(part 1 of 2)
# Autodesk Inventor assembly: carrier_board_2019-06-12
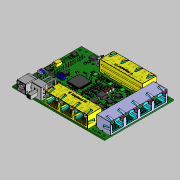
[picture p0: Inventor's stored thumbnail of the model, 180x180]
Saved by Autodesk Inventor 2020 (Build 240168000, 168)
## iProperties
Company: Open CASCADE
Created: 2019-06-12
Part Number: carrier_board_2019-06-12
Description: Open CASCADE Model
Document SubType Name: Assembly
Designer: Varga Daniel
Authority: Unknown
Title: Open CASCADE Shape Model
Author: Author
Sending System: Open CASCADE 6.8
Preprocessor: Open CASCADE STEP processor 6.8
## Documents named in this file (428)
- C:\!_Dani\!_cloud\OneDrive\!_munka\Revolution\StructuralParts\Brain\Inventor imported\BRpcbA\carrier_board_2019-06-12.iam
- C:\!_Dani\!_cloud\OneDrive\!_munka\Revolution\StructuralParts\Brain\Inventor imported\BRpcbA\Board.iam
- C:\!_Dani\!_cloud\OneDrive\!_munka\Revolution\StructuralParts\Brain\Inventor imported\BRpcbA\R177.iam
- C:\!_Dani\!_cloud\OneDrive\!_munka\Revolution\StructuralParts\Brain\Inventor imported\BRpcbA\CON1.iam
- C:\!_Dani\!_cloud\OneDrive\!_munka\Revolution\StructuralParts\Brain\Inventor imported\BRpcbA\R81.iam
- C:\!_Dani\!_cloud\OneDrive\!_munka\Revolution\StructuralParts\Brain\Inventor imported\BRpcbA\C45.iam
- C:\!_Dani\!_cloud\OneDrive\!_munka\Revolution\StructuralParts\Brain\Inventor imported\BRpcbA\U4.iam
- C:\!_Dani\!_cloud\OneDrive\!_munka\Revolution\StructuralParts\Brain\Inventor imported\BRpcbA\D37.iam
- C:\!_Dani\!_cloud\OneDrive\!_munka\Revolution\StructuralParts\Brain\Inventor imported\BRpcbA\D33.iam
- C:\!_Dani\!_cloud\OneDrive\!_munka\Revolution\StructuralParts\Brain\Inventor imported\BRpcbA\D32.iam
- C:\!_Dani\!_cloud\OneDrive\!_munka\Revolution\StructuralParts\Brain\Inventor imported\BRpcbA\C48.iam
- C:\!_Dani\!_cloud\OneDrive\!_munka\Revolution\StructuralParts\Brain\Inventor imported\BRpcbA\C47.iam
- C:\!_Dani\!_cloud\OneDrive\!_munka\Revolution\StructuralParts\Brain\Inventor imported\BRpcbA\D31.iam
- C:\!_Dani\!_cloud\OneDrive\!_munka\Revolution\StructuralParts\Brain\Inventor imported\BRpcbA\C46.iam
- C:\!_Dani\!_cloud\OneDrive\!_munka\Revolution\StructuralParts\Brain\Inventor imported\BRpcbA\R82.iam
- C:\!_Dani\!_cloud\OneDrive\!_munka\Revolution\StructuralParts\Brain\Inventor imported\BRpcbA\R26.iam
- C:\!_Dani\!_cloud\OneDrive\!_munka\Revolution\StructuralParts\Brain\Inventor imported\BRpcbA\C20.iam
- C:\!_Dani\!_cloud\OneDrive\!_munka\Revolution\StructuralParts\Brain\Inventor imported\BRpcbA\U2.iam
- C:\!_Dani\!_cloud\OneDrive\!_munka\Revolution\StructuralParts\Brain\Inventor imported\BRpcbA\D9.iam
- C:\!_Dani\!_cloud\OneDrive\!_munka\Revolution\StructuralParts\Brain\Inventor imported\BRpcbA\D5.iam
- C:\!_Dani\!_cloud\OneDrive\!_munka\Revolution\StructuralParts\Brain\Inventor imported\BRpcbA\D4.iam
- C:\!_Dani\!_cloud\OneDrive\!_munka\Revolution\StructuralParts\Brain\Inventor imported\BRpcbA\C23.iam
- C:\!_Dani\!_cloud\OneDrive\!_munka\Revolution\StructuralParts\Brain\Inventor imported\BRpcbA\C22.iam
- C:\!_Dani\!_cloud\OneDrive\!_munka\Revolution\StructuralParts\Brain\Inventor imported\BRpcbA\D1.iam
- C:\!_Dani\!_cloud\OneDrive\!_munka\Revolution\StructuralParts\Brain\Inventor imported\BRpcbA\C21.iam
- C:\!_Dani\!_cloud\OneDrive\!_munka\Revolution\StructuralParts\Brain\Inventor imported\BRpcbA\R27.iam
- C:\!_Dani\!_cloud\OneDrive\!_munka\Revolution\StructuralParts\Brain\Inventor imported\BRpcbA\R180.iam
- C:\!_Dani\!_cloud\OneDrive\!_munka\Revolution\StructuralParts\Brain\Inventor imported\BRpcbA\R109.iam
- C:\!_Dani\!_cloud\OneDrive\!_munka\Revolution\StructuralParts\Brain\Inventor imported\BRpcbA\R71.iam
- C:\!_Dani\!_cloud\OneDrive\!_munka\Revolution\StructuralParts\Brain\Inventor imported\BRpcbA\D72.iam
- C:\!_Dani\!_cloud\OneDrive\!_munka\Revolution\StructuralParts\Brain\Inventor imported\BRpcbA\Q4.iam
- C:\!_Dani\!_cloud\OneDrive\!_munka\Revolution\StructuralParts\Brain\Inventor imported\BRpcbA\R176.iam
- C:\!_Dani\!_cloud\OneDrive\!_munka\Revolution\StructuralParts\Brain\Inventor imported\BRpcbA\R175.iam
- C:\!_Dani\!_cloud\OneDrive\!_munka\Revolution\StructuralParts\Brain\Inventor imported\BRpcbA\R174.iam
- C:\!_Dani\!_cloud\OneDrive\!_munka\Revolution\StructuralParts\Brain\Inventor imported\BRpcbA\R173.iam
- C:\!_Dani\!_cloud\OneDrive\!_munka\Revolution\StructuralParts\Brain\Inventor imported\BRpcbA\R172.iam
- C:\!_Dani\!_cloud\OneDrive\!_munka\Revolution\StructuralParts\Brain\Inventor imported\BRpcbA\R171.iam
- C:\!_Dani\!_cloud\OneDrive\!_munka\Revolution\StructuralParts\Brain\Inventor imported\BRpcbA\R170.iam
- C:\!_Dani\!_cloud\OneDrive\!_munka\Revolution\StructuralParts\Brain\Inventor imported\BRpcbA\R169.iam
- C:\!_Dani\!_cloud\OneDrive\!_munka\Revolution\StructuralParts\Brain\Inventor imported\BRpcbA\R168.iam
- C:\!_Dani\!_cloud\OneDrive\!_munka\Revolution\StructuralParts\Brain\Inventor imported\BRpcbA\R167.iam
- C:\!_Dani\!_cloud\OneDrive\!_munka\Revolution\StructuralParts\Brain\Inventor imported\BRpcbA\R166.iam
- C:\!_Dani\!_cloud\OneDrive\!_munka\Revolution\StructuralParts\Brain\Inventor imported\BRpcbA\R165.iam
- C:\!_Dani\!_cloud\OneDrive\!_munka\Revolution\StructuralParts\Brain\Inventor imported\BRpcbA\R80.iam
- C:\!_Dani\!_cloud\OneDrive\!_munka\Revolution\StructuralParts\Brain\Inventor imported\BRpcbA\R79.iam
- C:\!_Dani\!_cloud\OneDrive\!_munka\Revolution\StructuralParts\Brain\Inventor imported\BRpcbA\R67.iam
- C:\!_Dani\!_cloud\OneDrive\!_munka\Revolution\StructuralParts\Brain\Inventor imported\BRpcbA\R66.iam
- C:\!_Dani\!_cloud\OneDrive\!_munka\Revolution\StructuralParts\Brain\Inventor imported\BRpcbA\R51.iam
- C:\!_Dani\!_cloud\OneDrive\!_munka\Revolution\StructuralParts\Brain\Inventor imported\BRpcbA\R50.iam
- C:\!_Dani\!_cloud\OneDrive\!_munka\Revolution\StructuralParts\Brain\Inventor imported\BRpcbA\R39.iam
- C:\!_Dani\!_cloud\OneDrive\!_munka\Revolution\StructuralParts\Brain\Inventor imported\BRpcbA\R38.iam
- C:\!_Dani\!_cloud\OneDrive\!_munka\Revolution\StructuralParts\Brain\Inventor imported\BRpcbA\R23.iam
- C:\!_Dani\!_cloud\OneDrive\!_munka\Revolution\StructuralParts\Brain\Inventor imported\BRpcbA\R22.iam
- C:\!_Dani\!_cloud\OneDrive\!_munka\Revolution\StructuralParts\Brain\Inventor imported\BRpcbA\R9.iam
- C:\!_Dani\!_cloud\OneDrive\!_munka\Revolution\StructuralParts\Brain\Inventor imported\BRpcbA\R8.iam
- C:\!_Dani\!_cloud\OneDrive\!_munka\Revolution\StructuralParts\Brain\Inventor imported\BRpcbA\FB1.iam
- C:\!_Dani\!_cloud\OneDrive\!_munka\Revolution\StructuralParts\Brain\Inventor imported\BRpcbA\C2.iam
- C:\!_Dani\!_cloud\OneDrive\!_munka\Revolution\StructuralParts\Brain\Inventor imported\BRpcbA\FU1.iam
- C:\!_Dani\!_cloud\OneDrive\!_munka\Revolution\StructuralParts\Brain\Inventor imported\BRpcbA\C97.iam
- C:\!_Dani\!_cloud\OneDrive\!_munka\Revolution\StructuralParts\Brain\Inventor imported\BRpcbA\U16.iam
- C:\!_Dani\!_cloud\OneDrive\!_munka\Revolution\StructuralParts\Brain\Inventor imported\BRpcbA\U14.iam
- C:\!_Dani\!_cloud\OneDrive\!_munka\Revolution\StructuralParts\Brain\Inventor imported\BRpcbA\U8.iam
- C:\!_Dani\!_cloud\OneDrive\!_munka\Revolution\StructuralParts\Brain\Inventor imported\BRpcbA\U6.iam
- C:\!_Dani\!_cloud\OneDrive\!_munka\Revolution\StructuralParts\Brain\Inventor imported\BRpcbA\R161.iam
- C:\!_Dani\!_cloud\OneDrive\!_munka\Revolution\StructuralParts\Brain\Inventor imported\BRpcbA\R150.iam
- C:\!_Dani\!_cloud\OneDrive\!_munka\Revolution\StructuralParts\Brain\Inventor imported\BRpcbA\R127.iam
- C:\!_Dani\!_cloud\OneDrive\!_munka\Revolution\StructuralParts\Brain\Inventor imported\BRpcbA\R118.iam
- C:\!_Dani\!_cloud\OneDrive\!_munka\Revolution\StructuralParts\Brain\Inventor imported\BRpcbA\R116.iam
- C:\!_Dani\!_cloud\OneDrive\!_munka\Revolution\StructuralParts\Brain\Inventor imported\BRpcbA\R115.iam
- C:\!_Dani\!_cloud\OneDrive\!_munka\Revolution\StructuralParts\Brain\Inventor imported\BRpcbA\R114.iam
- C:\!_Dani\!_cloud\OneDrive\!_munka\Revolution\StructuralParts\Brain\Inventor imported\BRpcbA\R111.iam
- C:\!_Dani\!_cloud\OneDrive\!_munka\Revolution\StructuralParts\Brain\Inventor imported\BRpcbA\R110.iam
- C:\!_Dani\!_cloud\OneDrive\!_munka\Revolution\StructuralParts\Brain\Inventor imported\BRpcbA\R106.iam
- C:\!_Dani\!_cloud\OneDrive\!_munka\Revolution\StructuralParts\Brain\Inventor imported\BRpcbA\R105.iam
- C:\!_Dani\!_cloud\OneDrive\!_munka\Revolution\StructuralParts\Brain\Inventor imported\BRpcbA\R99.iam
- C:\!_Dani\!_cloud\OneDrive\!_munka\Revolution\StructuralParts\Brain\Inventor imported\BRpcbA\R98.iam
- C:\!_Dani\!_cloud\OneDrive\!_munka\Revolution\StructuralParts\Brain\Inventor imported\BRpcbA\R95.iam
- C:\!_Dani\!_cloud\OneDrive\!_munka\Revolution\StructuralParts\Brain\Inventor imported\BRpcbA\R92.iam
- C:\!_Dani\!_cloud\OneDrive\!_munka\Revolution\StructuralParts\Brain\Inventor imported\BRpcbA\R89.iam
- C:\!_Dani\!_cloud\OneDrive\!_munka\Revolution\StructuralParts\Brain\Inventor imported\BRpcbA\R88.iam
- C:\!_Dani\!_cloud\OneDrive\!_munka\Revolution\StructuralParts\Brain\Inventor imported\BRpcbA\R74.iam
- C:\!_Dani\!_cloud\OneDrive\!_munka\Revolution\StructuralParts\Brain\Inventor imported\BRpcbA\R68.iam
- C:\!_Dani\!_cloud\OneDrive\!_munka\Revolution\StructuralParts\Brain\Inventor imported\BRpcbA\R54.iam
- C:\!_Dani\!_cloud\OneDrive\!_munka\Revolution\StructuralParts\Brain\Inventor imported\BRpcbA\R47.iam
- C:\!_Dani\!_cloud\OneDrive\!_munka\Revolution\StructuralParts\Brain\Inventor imported\BRpcbA\R46.iam
- C:\!_Dani\!_cloud\OneDrive\!_munka\Revolution\StructuralParts\Brain\Inventor imported\BRpcbA\R45.iam
- C:\!_Dani\!_cloud\OneDrive\!_munka\Revolution\StructuralParts\Brain\Inventor imported\BRpcbA\R41.iam
- C:\!_Dani\!_cloud\OneDrive\!_munka\Revolution\StructuralParts\Brain\Inventor imported\BRpcbA\R32.iam
- C:\!_Dani\!_cloud\OneDrive\!_munka\Revolution\StructuralParts\Brain\Inventor imported\BRpcbA\R31.iam
- C:\!_Dani\!_cloud\OneDrive\!_munka\Revolution\StructuralParts\Brain\Inventor imported\BRpcbA\R29.iam
- C:\!_Dani\!_cloud\OneDrive\!_munka\Revolution\StructuralParts\Brain\Inventor imported\BRpcbA\R28.iam
- C:\!_Dani\!_cloud\OneDrive\!_munka\Revolution\StructuralParts\Brain\Inventor imported\BRpcbA\R19.iam
- C:\!_Dani\!_cloud\OneDrive\!_munka\Revolution\StructuralParts\Brain\Inventor imported\BRpcbA\R15.iam
- C:\!_Dani\!_cloud\OneDrive\!_munka\Revolution\StructuralParts\Brain\Inventor imported\BRpcbA\R12.iam
- C:\!_Dani\!_cloud\OneDrive\!_munka\Revolution\StructuralParts\Brain\Inventor imported\BRpcbA\R2.iam
- C:\!_Dani\!_cloud\OneDrive\!_munka\Revolution\StructuralParts\Brain\Inventor imported\BRpcbA\L4.iam
- C:\!_Dani\!_cloud\OneDrive\!_munka\Revolution\StructuralParts\Brain\Inventor imported\BRpcbA\FU21.iam
- C:\!_Dani\!_cloud\OneDrive\!_munka\Revolution\StructuralParts\Brain\Inventor imported\BRpcbA\FB11.iam
- C:\!_Dani\!_cloud\OneDrive\!_munka\Revolution\StructuralParts\Brain\Inventor imported\BRpcbA\FB9.iam
- C:\!_Dani\!_cloud\OneDrive\!_munka\Revolution\StructuralParts\Brain\Inventor imported\BRpcbA\FB7.iam
- C:\!_Dani\!_cloud\OneDrive\!_munka\Revolution\StructuralParts\Brain\Inventor imported\BRpcbA\FB5.iam
- C:\!_Dani\!_cloud\OneDrive\!_munka\Revolution\StructuralParts\Brain\Inventor imported\BRpcbA\D55.iam
- C:\!_Dani\!_cloud\OneDrive\!_munka\Revolution\StructuralParts\Brain\Inventor imported\BRpcbA\D53.iam
- C:\!_Dani\!_cloud\OneDrive\!_munka\Revolution\StructuralParts\Brain\Inventor imported\BRpcbA\D52.iam
- C:\!_Dani\!_cloud\OneDrive\!_munka\Revolution\StructuralParts\Brain\Inventor imported\BRpcbA\D51.iam
- C:\!_Dani\!_cloud\OneDrive\!_munka\Revolution\StructuralParts\Brain\Inventor imported\BRpcbA\D48.iam
- C:\!_Dani\!_cloud\OneDrive\!_munka\Revolution\StructuralParts\Brain\Inventor imported\BRpcbA\D43.iam
- C:\!_Dani\!_cloud\OneDrive\!_munka\Revolution\StructuralParts\Brain\Inventor imported\BRpcbA\D42.iam
- C:\!_Dani\!_cloud\OneDrive\!_munka\Revolution\StructuralParts\Brain\Inventor imported\BRpcbA\D38.iam
- C:\!_Dani\!_cloud\OneDrive\!_munka\Revolution\StructuralParts\Brain\Inventor imported\BRpcbA\D26.iam
- C:\!_Dani\!_cloud\OneDrive\!_munka\Revolution\StructuralParts\Brain\Inventor imported\BRpcbA\D15.iam
- C:\!_Dani\!_cloud\OneDrive\!_munka\Revolution\StructuralParts\Brain\Inventor imported\BRpcbA\D11.iam
- C:\!_Dani\!_cloud\OneDrive\!_munka\Revolution\StructuralParts\Brain\Inventor imported\BRpcbA\D7.iam
- C:\!_Dani\!_cloud\OneDrive\!_munka\Revolution\StructuralParts\Brain\Inventor imported\BRpcbA\D6.iam
- C:\!_Dani\!_cloud\OneDrive\!_munka\Revolution\StructuralParts\Brain\Inventor imported\BRpcbA\D3.iam
- C:\!_Dani\!_cloud\OneDrive\!_munka\Revolution\StructuralParts\Brain\Inventor imported\BRpcbA\C117.iam
- C:\!_Dani\!_cloud\OneDrive\!_munka\Revolution\StructuralParts\Brain\Inventor imported\BRpcbA\C116.iam
- C:\!_Dani\!_cloud\OneDrive\!_munka\Revolution\StructuralParts\Brain\Inventor imported\BRpcbA\C115.iam
- C:\!_Dani\!_cloud\OneDrive\!_munka\Revolution\StructuralParts\Brain\Inventor imported\BRpcbA\C114.iam
- C:\!_Dani\!_cloud\OneDrive\!_munka\Revolution\StructuralParts\Brain\Inventor imported\BRpcbA\C113.iam
- C:\!_Dani\!_cloud\OneDrive\!_munka\Revolution\StructuralParts\Brain\Inventor imported\BRpcbA\C101.iam
- C:\!_Dani\!_cloud\OneDrive\!_munka\Revolution\StructuralParts\Brain\Inventor imported\BRpcbA\C91.iam
- C:\!_Dani\!_cloud\OneDrive\!_munka\Revolution\StructuralParts\Brain\Inventor imported\BRpcbA\C85.iam
- C:\!_Dani\!_cloud\OneDrive\!_munka\Revolution\StructuralParts\Brain\Inventor imported\BRpcbA\C80.iam
- C:\!_Dani\!_cloud\OneDrive\!_munka\Revolution\StructuralParts\Brain\Inventor imported\BRpcbA\C78.iam
- C:\!_Dani\!_cloud\OneDrive\!_munka\Revolution\StructuralParts\Brain\Inventor imported\BRpcbA\C77.iam
- C:\!_Dani\!_cloud\OneDrive\!_munka\Revolution\StructuralParts\Brain\Inventor imported\BRpcbA\C76.iam
- C:\!_Dani\!_cloud\OneDrive\!_munka\Revolution\StructuralParts\Brain\Inventor imported\BRpcbA\C75.iam
- C:\!_Dani\!_cloud\OneDrive\!_munka\Revolution\StructuralParts\Brain\Inventor imported\BRpcbA\C72.iam
- C:\!_Dani\!_cloud\OneDrive\!_munka\Revolution\StructuralParts\Brain\Inventor imported\BRpcbA\C70.iam
- C:\!_Dani\!_cloud\OneDrive\!_munka\Revolution\StructuralParts\Brain\Inventor imported\BRpcbA\C58.iam
- C:\!_Dani\!_cloud\OneDrive\!_munka\Revolution\StructuralParts\Brain\Inventor imported\BRpcbA\C55.iam
- C:\!_Dani\!_cloud\OneDrive\!_munka\Revolution\StructuralParts\Brain\Inventor imported\BRpcbA\C37.iam
- C:\!_Dani\!_cloud\OneDrive\!_munka\Revolution\StructuralParts\Brain\Inventor imported\BRpcbA\C32.iam
- C:\!_Dani\!_cloud\OneDrive\!_munka\Revolution\StructuralParts\Brain\Inventor imported\BRpcbA\C29.iam
- C:\!_Dani\!_cloud\OneDrive\!_munka\Revolution\StructuralParts\Brain\Inventor imported\BRpcbA\R108.iam
- C:\!_Dani\!_cloud\OneDrive\!_munka\Revolution\StructuralParts\Brain\Inventor imported\BRpcbA\R107.iam
- C:\!_Dani\!_cloud\OneDrive\!_munka\Revolution\StructuralParts\Brain\Inventor imported\BRpcbA\D46.iam
- C:\!_Dani\!_cloud\OneDrive\!_munka\Revolution\StructuralParts\Brain\Inventor imported\BRpcbA\C71.iam
- C:\!_Dani\!_cloud\OneDrive\!_munka\Revolution\StructuralParts\Brain\Inventor imported\BRpcbA\D71.iam
- C:\!_Dani\!_cloud\OneDrive\!_munka\Revolution\StructuralParts\Brain\Inventor imported\BRpcbA\D70.iam
- C:\!_Dani\!_cloud\OneDrive\!_munka\Revolution\StructuralParts\Brain\Inventor imported\BRpcbA\D69.iam
- C:\!_Dani\!_cloud\OneDrive\!_munka\Revolution\StructuralParts\Brain\Inventor imported\BRpcbA\D68.iam
- C:\!_Dani\!_cloud\OneDrive\!_munka\Revolution\StructuralParts\Brain\Inventor imported\BRpcbA\D66.iam
- C:\!_Dani\!_cloud\OneDrive\!_munka\Revolution\StructuralParts\Brain\Inventor imported\BRpcbA\D65.iam
- C:\!_Dani\!_cloud\OneDrive\!_munka\Revolution\StructuralParts\Brain\Inventor imported\BRpcbA\D64.iam
- C:\!_Dani\!_cloud\OneDrive\!_munka\Revolution\StructuralParts\Brain\Inventor imported\BRpcbA\D61.iam
- C:\!_Dani\!_cloud\OneDrive\!_munka\Revolution\StructuralParts\Brain\Inventor imported\BRpcbA\D60.iam
- C:\!_Dani\!_cloud\OneDrive\!_munka\Revolution\StructuralParts\Brain\Inventor imported\BRpcbA\D17.iam
- C:\!_Dani\!_cloud\OneDrive\!_munka\Revolution\StructuralParts\Brain\Inventor imported\BRpcbA\R148.iam
- C:\!_Dani\!_cloud\OneDrive\!_munka\Revolution\StructuralParts\Brain\Inventor imported\BRpcbA\D58.iam
- C:\!_Dani\!_cloud\OneDrive\!_munka\Revolution\StructuralParts\Brain\Inventor imported\BRpcbA\D56.iam
- C:\!_Dani\!_cloud\OneDrive\!_munka\Revolution\StructuralParts\Brain\Inventor imported\BRpcbA\D24.iam
- C:\!_Dani\!_cloud\OneDrive\!_munka\Revolution\StructuralParts\Brain\Inventor imported\BRpcbA\D63.iam
- C:\!_Dani\!_cloud\OneDrive\!_munka\Revolution\StructuralParts\Brain\Inventor imported\BRpcbA\D67.iam
- C:\!_Dani\!_cloud\OneDrive\!_munka\Revolution\StructuralParts\Brain\Inventor imported\BRpcbA\Q16.iam
- C:\!_Dani\!_cloud\OneDrive\!_munka\Revolution\StructuralParts\Brain\Inventor imported\BRpcbA\Q17.iam
- C:\!_Dani\!_cloud\OneDrive\!_munka\Revolution\StructuralParts\Brain\Inventor imported\BRpcbA\R153.iam
- C:\!_Dani\!_cloud\OneDrive\!_munka\Revolution\StructuralParts\Brain\Inventor imported\BRpcbA\R156.iam
- C:\!_Dani\!_cloud\OneDrive\!_munka\Revolution\StructuralParts\Brain\Inventor imported\BRpcbA\R139.iam
- C:\!_Dani\!_cloud\OneDrive\!_munka\Revolution\StructuralParts\Brain\Inventor imported\BRpcbA\R144.iam
- C:\!_Dani\!_cloud\OneDrive\!_munka\Revolution\StructuralParts\Brain\Inventor imported\BRpcbA\R141.iam
- C:\!_Dani\!_cloud\OneDrive\!_munka\Revolution\StructuralParts\Brain\Inventor imported\BRpcbA\Q15.iam
- C:\!_Dani\!_cloud\OneDrive\!_munka\Revolution\StructuralParts\Brain\Inventor imported\BRpcbA\Q14.iam
- C:\!_Dani\!_cloud\OneDrive\!_munka\Revolution\StructuralParts\Brain\Inventor imported\BRpcbA\D62.iam
- C:\!_Dani\!_cloud\OneDrive\!_munka\Revolution\StructuralParts\Brain\Inventor imported\BRpcbA\D59.iam
- C:\!_Dani\!_cloud\OneDrive\!_munka\Revolution\StructuralParts\Brain\Inventor imported\BRpcbA\D54.iam
- C:\!_Dani\!_cloud\OneDrive\!_munka\Revolution\StructuralParts\Brain\Inventor imported\BRpcbA\D57.iam
- C:\!_Dani\!_cloud\OneDrive\!_munka\Revolution\StructuralParts\Brain\Inventor imported\BRpcbA\Q12.iam
- C:\!_Dani\!_cloud\OneDrive\!_munka\Revolution\StructuralParts\Brain\Inventor imported\BRpcbA\Q13.iam
- C:\!_Dani\!_cloud\OneDrive\!_munka\Revolution\StructuralParts\Brain\Inventor imported\BRpcbA\R131.iam
- C:\!_Dani\!_cloud\OneDrive\!_munka\Revolution\StructuralParts\Brain\Inventor imported\BRpcbA\R132.iam
- C:\!_Dani\!_cloud\OneDrive\!_munka\Revolution\StructuralParts\Brain\Inventor imported\BRpcbA\C42.iam
- C:\!_Dani\!_cloud\OneDrive\!_munka\Revolution\StructuralParts\Brain\Inventor imported\BRpcbA\C33.iam
- C:\!_Dani\!_cloud\OneDrive\!_munka\Revolution\StructuralParts\Brain\Inventor imported\BRpcbA\R58.iam
- C:\!_Dani\!_cloud\OneDrive\!_munka\Revolution\StructuralParts\Brain\Inventor imported\BRpcbA\R55.iam
- C:\!_Dani\!_cloud\OneDrive\!_munka\Revolution\StructuralParts\Brain\Inventor imported\BRpcbA\R48.iam
- C:\!_Dani\!_cloud\OneDrive\!_munka\Revolution\StructuralParts\Brain\Inventor imported\BRpcbA\R34.iam
- C:\!_Dani\!_cloud\OneDrive\!_munka\Revolution\StructuralParts\Brain\Inventor imported\BRpcbA\R49.iam
- C:\!_Dani\!_cloud\OneDrive\!_munka\Revolution\StructuralParts\Brain\Inventor imported\BRpcbA\Q5.iam
- C:\!_Dani\!_cloud\OneDrive\!_munka\Revolution\StructuralParts\Brain\Inventor imported\BRpcbA\FU8.iam
- C:\!_Dani\!_cloud\OneDrive\!_munka\Revolution\StructuralParts\Brain\Inventor imported\BRpcbA\FU7.iam
- C:\!_Dani\!_cloud\OneDrive\!_munka\Revolution\StructuralParts\Brain\Inventor imported\BRpcbA\D36.iam
- C:\!_Dani\!_cloud\OneDrive\!_munka\Revolution\StructuralParts\Brain\Inventor imported\BRpcbA\D35.iam
- C:\!_Dani\!_cloud\OneDrive\!_munka\Revolution\StructuralParts\Brain\Inventor imported\BRpcbA\D34.iam
- C:\!_Dani\!_cloud\OneDrive\!_munka\Revolution\StructuralParts\Brain\Inventor imported\BRpcbA\C63.iam
- C:\!_Dani\!_cloud\OneDrive\!_munka\Revolution\StructuralParts\Brain\Inventor imported\BRpcbA\C36.iam
- C:\!_Dani\!_cloud\OneDrive\!_munka\Revolution\StructuralParts\Brain\Inventor imported\BRpcbA\C35.iam
- C:\!_Dani\!_cloud\OneDrive\!_munka\Revolution\StructuralParts\Brain\Inventor imported\BRpcbA\C39.iam
- C:\!_Dani\!_cloud\OneDrive\!_munka\Revolution\StructuralParts\Brain\Inventor imported\BRpcbA\C40.iam
- C:\!_Dani\!_cloud\OneDrive\!_munka\Revolution\StructuralParts\Brain\Inventor imported\BRpcbA\C79.iam
- C:\!_Dani\!_cloud\OneDrive\!_munka\Revolution\StructuralParts\Brain\Inventor imported\BRpcbA\C81.iam
- C:\!_Dani\!_cloud\OneDrive\!_munka\Revolution\StructuralParts\Brain\Inventor imported\BRpcbA\D39.iam
- C:\!_Dani\!_cloud\OneDrive\!_munka\Revolution\StructuralParts\Brain\Inventor imported\BRpcbA\D40.iam
- C:\!_Dani\!_cloud\OneDrive\!_munka\Revolution\StructuralParts\Brain\Inventor imported\BRpcbA\D41.iam
- C:\!_Dani\!_cloud\OneDrive\!_munka\Revolution\StructuralParts\Brain\Inventor imported\BRpcbA\FU10.iam
- C:\!_Dani\!_cloud\OneDrive\!_munka\Revolution\StructuralParts\Brain\Inventor imported\BRpcbA\FU9.iam
- C:\!_Dani\!_cloud\OneDrive\!_munka\Revolution\StructuralParts\Brain\Inventor imported\BRpcbA\Q6.iam
- C:\!_Dani\!_cloud\OneDrive\!_munka\Revolution\StructuralParts\Brain\Inventor imported\BRpcbA\R63.iam
- C:\!_Dani\!_cloud\OneDrive\!_munka\Revolution\StructuralParts\Brain\Inventor imported\BRpcbA\R70.iam
- C:\!_Dani\!_cloud\OneDrive\!_munka\Revolution\StructuralParts\Brain\Inventor imported\BRpcbA\R42.iam
- C:\!_Dani\!_cloud\OneDrive\!_munka\Revolution\StructuralParts\Brain\Inventor imported\BRpcbA\R43.iam
- C:\!_Dani\!_cloud\OneDrive\!_munka\Revolution\StructuralParts\Brain\Inventor imported\BRpcbA\R61.iam
- C:\!_Dani\!_cloud\OneDrive\!_munka\Revolution\StructuralParts\Brain\Inventor imported\BRpcbA\R64.iam
- C:\!_Dani\!_cloud\OneDrive\!_munka\Revolution\StructuralParts\Brain\Inventor imported\BRpcbA\C28.iam
- C:\!_Dani\!_cloud\OneDrive\!_munka\Revolution\StructuralParts\Brain\Inventor imported\BRpcbA\C24.iam
- C:\!_Dani\!_cloud\OneDrive\!_munka\Revolution\StructuralParts\Brain\Inventor imported\BRpcbA\C34.iam
- C:\!_Dani\!_cloud\OneDrive\!_munka\Revolution\StructuralParts\Brain\Inventor imported\BRpcbA\C73.iam
- C:\!_Dani\!_cloud\OneDrive\!_munka\Revolution\StructuralParts\Brain\Inventor imported\BRpcbA\D18.iam
- C:\!_Dani\!_cloud\OneDrive\!_munka\Revolution\StructuralParts\Brain\Inventor imported\BRpcbA\D19.iam
- C:\!_Dani\!_cloud\OneDrive\!_munka\Revolution\StructuralParts\Brain\Inventor imported\BRpcbA\D23.iam
- C:\!_Dani\!_cloud\OneDrive\!_munka\Revolution\StructuralParts\Brain\Inventor imported\BRpcbA\U3.iam
- C:\!_Dani\!_cloud\OneDrive\!_munka\Revolution\StructuralParts\Brain\Inventor imported\BRpcbA\U5.iam
- C:\!_Dani\!_cloud\OneDrive\!_munka\Revolution\StructuralParts\Brain\Inventor imported\BRpcbA\R36.iam
- C:\!_Dani\!_cloud\OneDrive\!_munka\Revolution\StructuralParts\Brain\Inventor imported\BRpcbA\R33.iam
- C:\!_Dani\!_cloud\OneDrive\!_munka\Revolution\StructuralParts\Brain\Inventor imported\BRpcbA\FU6.iam
- C:\!_Dani\!_cloud\OneDrive\!_munka\Revolution\StructuralParts\Brain\Inventor imported\BRpcbA\FU5.iam
- C:\!_Dani\!_cloud\OneDrive\!_munka\Revolution\StructuralParts\Brain\Inventor imported\BRpcbA\D14.iam
- C:\!_Dani\!_cloud\OneDrive\!_munka\Revolution\StructuralParts\Brain\Inventor imported\BRpcbA\D13.iam
- C:\!_Dani\!_cloud\OneDrive\!_munka\Revolution\StructuralParts\Brain\Inventor imported\BRpcbA\D12.iam
- C:\!_Dani\!_cloud\OneDrive\!_munka\Revolution\StructuralParts\Brain\Inventor imported\BRpcbA\C53.iam
- C:\!_Dani\!_cloud\OneDrive\!_munka\Revolution\StructuralParts\Brain\Inventor imported\BRpcbA\C31.iam
- C:\!_Dani\!_cloud\OneDrive\!_munka\Revolution\StructuralParts\Brain\Inventor imported\BRpcbA\C30.iam
- C:\!_Dani\!_cloud\OneDrive\!_munka\Revolution\StructuralParts\Brain\Inventor imported\BRpcbA\C26.iam
- C:\!_Dani\!_cloud\OneDrive\!_munka\Revolution\StructuralParts\Brain\Inventor imported\BRpcbA\C27.iam
- C:\!_Dani\!_cloud\OneDrive\!_munka\Revolution\StructuralParts\Brain\Inventor imported\BRpcbA\R25.iam
- C:\!_Dani\!_cloud\OneDrive\!_munka\Revolution\StructuralParts\Brain\Inventor imported\BRpcbA\R17.iam
- C:\!_Dani\!_cloud\OneDrive\!_munka\Revolution\StructuralParts\Brain\Inventor imported\BRpcbA\C19.iam
- C:\!_Dani\!_cloud\OneDrive\!_munka\Revolution\StructuralParts\Brain\Inventor imported\BRpcbA\C18.iam
- C:\!_Dani\!_cloud\OneDrive\!_munka\Revolution\StructuralParts\Brain\Inventor imported\BRpcbA\C25.iam
- C:\!_Dani\!_cloud\OneDrive\!_munka\Revolution\StructuralParts\Brain\Inventor imported\BRpcbA\C51.iam
- C:\!_Dani\!_cloud\OneDrive\!_munka\Revolution\StructuralParts\Brain\Inventor imported\BRpcbA\D10.iam
- C:\!_Dani\!_cloud\OneDrive\!_munka\Revolution\StructuralParts\Brain\Inventor imported\BRpcbA\D8.iam
- C:\!_Dani\!_cloud\OneDrive\!_munka\Revolution\StructuralParts\Brain\Inventor imported\BRpcbA\FU3.iam
- C:\!_Dani\!_cloud\OneDrive\!_munka\Revolution\StructuralParts\Brain\Inventor imported\BRpcbA\FU4.iam
- C:\!_Dani\!_cloud\OneDrive\!_munka\Revolution\StructuralParts\Brain\Inventor imported\BRpcbA\Q3.iam
- C:\!_Dani\!_cloud\OneDrive\!_munka\Revolution\StructuralParts\Brain\Inventor imported\BRpcbA\R21.iam
- C:\!_Dani\!_cloud\OneDrive\!_munka\Revolution\StructuralParts\Brain\Inventor imported\BRpcbA\R30.iam
- C:\!_Dani\!_cloud\OneDrive\!_munka\Revolution\StructuralParts\Brain\Inventor imported\BRpcbA\R16.iam
- C:\!_Dani\!_cloud\OneDrive\!_munka\Revolution\StructuralParts\Brain\Inventor imported\BRpcbA\R20.iam
- C:\!_Dani\!_cloud\OneDrive\!_munka\Revolution\StructuralParts\Brain\Inventor imported\BRpcbA\R24.iam
- C:\!_Dani\!_cloud\OneDrive\!_munka\Revolution\StructuralParts\Brain\Inventor imported\BRpcbA\R160.iam
- C:\!_Dani\!_cloud\OneDrive\!_munka\Revolution\StructuralParts\Brain\Inventor imported\BRpcbA\C100.iam
- C:\!_Dani\!_cloud\OneDrive\!_munka\Revolution\StructuralParts\Brain\Inventor imported\BRpcbA\C102.iam
- C:\!_Dani\!_cloud\OneDrive\!_munka\Revolution\StructuralParts\Brain\Inventor imported\BRpcbA\C110.iam
- C:\!_Dani\!_cloud\OneDrive\!_munka\Revolution\StructuralParts\Brain\Inventor imported\BRpcbA\D27.iam
- C:\!_Dani\!_cloud\OneDrive\!_munka\Revolution\StructuralParts\Brain\Inventor imported\BRpcbA\D28.iam
- C:\!_Dani\!_cloud\OneDrive\!_munka\Revolution\StructuralParts\Brain\Inventor imported\BRpcbA\FB10.iam
- C:\!_Dani\!_cloud\OneDrive\!_munka\Revolution\StructuralParts\Brain\Inventor imported\BRpcbA\FU19.iam
- C:\!_Dani\!_cloud\OneDrive\!_munka\Revolution\StructuralParts\Brain\Inventor imported\BRpcbA\FU20.iam
- C:\!_Dani\!_cloud\OneDrive\!_munka\Revolution\StructuralParts\Brain\Inventor imported\BRpcbA\R154.iam
- C:\!_Dani\!_cloud\OneDrive\!_munka\Revolution\StructuralParts\Brain\Inventor imported\BRpcbA\R155.iam
- C:\!_Dani\!_cloud\OneDrive\!_munka\Revolution\StructuralParts\Brain\Inventor imported\BRpcbA\R159.iam
- C:\!_Dani\!_cloud\OneDrive\!_munka\Revolution\StructuralParts\Brain\Inventor imported\BRpcbA\R151.iam
- C:\!_Dani\!_cloud\OneDrive\!_munka\Revolution\StructuralParts\Brain\Inventor imported\BRpcbA\R158.iam
- C:\!_Dani\!_cloud\OneDrive\!_munka\Revolution\StructuralParts\Brain\Inventor imported\BRpcbA\R181.iam
- C:\!_Dani\!_cloud\OneDrive\!_munka\Revolution\StructuralParts\Brain\Inventor imported\BRpcbA\D21.iam
- C:\!_Dani\!_cloud\OneDrive\!_munka\Revolution\StructuralParts\Brain\Inventor imported\BRpcbA\R157.iam
- C:\!_Dani\!_cloud\OneDrive\!_munka\Revolution\StructuralParts\Brain\Inventor imported\BRpcbA\R128.iam
- C:\!_Dani\!_cloud\OneDrive\!_munka\Revolution\StructuralParts\Brain\Inventor imported\BRpcbA\R129.iam
- C:\!_Dani\!_cloud\OneDrive\!_munka\Revolution\StructuralParts\Brain\Inventor imported\BRpcbA\R126.iam
- C:\!_Dani\!_cloud\OneDrive\!_munka\Revolution\StructuralParts\Brain\Inventor imported\BRpcbA\R125.iam
- C:\!_Dani\!_cloud\OneDrive\!_munka\Revolution\StructuralParts\Brain\Inventor imported\BRpcbA\R123.iam
- C:\!_Dani\!_cloud\OneDrive\!_munka\Revolution\StructuralParts\Brain\Inventor imported\BRpcbA\FU14.iam
- C:\!_Dani\!_cloud\OneDrive\!_munka\Revolution\StructuralParts\Brain\Inventor imported\BRpcbA\FU13.iam
- C:\!_Dani\!_cloud\OneDrive\!_munka\Revolution\StructuralParts\Brain\Inventor imported\BRpcbA\FB4.iam
- C:\!_Dani\!_cloud\OneDrive\!_munka\Revolution\StructuralParts\Brain\Inventor imported\BRpcbA\C104.iam
- C:\!_Dani\!_cloud\OneDrive\!_munka\Revolution\StructuralParts\Brain\Inventor imported\BRpcbA\C86.iam
- C:\!_Dani\!_cloud\OneDrive\!_munka\Revolution\StructuralParts\Brain\Inventor imported\BRpcbA\C84.iam
- C:\!_Dani\!_cloud\OneDrive\!_munka\Revolution\StructuralParts\Brain\Inventor imported\BRpcbA\C88.iam
- C:\!_Dani\!_cloud\OneDrive\!_munka\Revolution\StructuralParts\Brain\Inventor imported\BRpcbA\C90.iam
- C:\!_Dani\!_cloud\OneDrive\!_munka\Revolution\StructuralParts\Brain\Inventor imported\BRpcbA\C103.iam
- C:\!_Dani\!_cloud\OneDrive\!_munka\Revolution\StructuralParts\Brain\Inventor imported\BRpcbA\C108.iam
- C:\!_Dani\!_cloud\OneDrive\!_munka\Revolution\StructuralParts\Brain\Inventor imported\BRpcbA\D20.iam
- C:\!_Dani\!_cloud\OneDrive\!_munka\Revolution\StructuralParts\Brain\Inventor imported\BRpcbA\D22.iam
- C:\!_Dani\!_cloud\OneDrive\!_munka\Revolution\StructuralParts\Brain\Inventor imported\BRpcbA\FB6.iam
- C:\!_Dani\!_cloud\OneDrive\!_munka\Revolution\StructuralParts\Brain\Inventor imported\BRpcbA\FU15.iam
- C:\!_Dani\!_cloud\OneDrive\!_munka\Revolution\StructuralParts\Brain\Inventor imported\BRpcbA\FU16.iam
- C:\!_Dani\!_cloud\OneDrive\!_munka\Revolution\StructuralParts\Brain\Inventor imported\BRpcbA\R135.iam
- C:\!_Dani\!_cloud\OneDrive\!_munka\Revolution\StructuralParts\Brain\Inventor imported\BRpcbA\R136.iam
- C:\!_Dani\!_cloud\OneDrive\!_munka\Revolution\StructuralParts\Brain\Inventor imported\BRpcbA\R133.iam
- C:\!_Dani\!_cloud\OneDrive\!_munka\Revolution\StructuralParts\Brain\Inventor imported\BRpcbA\R138.iam
- C:\!_Dani\!_cloud\OneDrive\!_munka\Revolution\StructuralParts\Brain\Inventor imported\BRpcbA\R137.iam
- C:\!_Dani\!_cloud\OneDrive\!_munka\Revolution\StructuralParts\Brain\Inventor imported\BRpcbA\R163.iam
- C:\!_Dani\!_cloud\OneDrive\!_munka\Revolution\StructuralParts\Brain\Inventor imported\BRpcbA\CON2.iam
- C:\!_Dani\!_cloud\OneDrive\!_munka\Revolution\StructuralParts\Brain\Inventor imported\BRpcbA\U11.iam
- C:\!_Dani\!_cloud\OneDrive\!_munka\Revolution\StructuralParts\Brain\Inventor imported\BRpcbA\U10.iam
- C:\!_Dani\!_cloud\OneDrive\!_munka\Revolution\StructuralParts\Brain\Inventor imported\BRpcbA\U7.iam
- C:\!_Dani\!_cloud\OneDrive\!_munka\Revolution\StructuralParts\Brain\Inventor imported\BRpcbA\U20.iam
- C:\!_Dani\!_cloud\OneDrive\!_munka\Revolution\StructuralParts\Brain\Inventor imported\BRpcbA\U19.iam
- C:\!_Dani\!_cloud\OneDrive\!_munka\Revolution\StructuralParts\Brain\Inventor imported\BRpcbA\U18.iam
- C:\!_Dani\!_cloud\OneDrive\!_munka\Revolution\StructuralParts\Brain\Inventor imported\BRpcbA\U17.iam
- C:\!_Dani\!_cloud\OneDrive\!_munka\Revolution\StructuralParts\Brain\Inventor imported\BRpcbA\U1.iam
- C:\!_Dani\!_cloud\OneDrive\!_munka\Revolution\StructuralParts\Brain\Inventor imported\BRpcbA\S1.iam
- C:\!_Dani\!_cloud\OneDrive\!_munka\Revolution\StructuralParts\Brain\Inventor imported\BRpcbA\R6.iam
- C:\!_Dani\!_cloud\OneDrive\!_munka\Revolution\StructuralParts\Brain\Inventor imported\BRpcbA\R162.iam
- C:\!_Dani\!_cloud\OneDrive\!_munka\Revolution\StructuralParts\Brain\Inventor imported\BRpcbA\R152.iam
- C:\!_Dani\!_cloud\OneDrive\!_munka\Revolution\StructuralParts\Brain\Inventor imported\BRpcbA\R164.iam
- C:\!_Dani\!_cloud\OneDrive\!_munka\Revolution\StructuralParts\Brain\Inventor imported\BRpcbA\R147.iam
- C:\!_Dani\!_cloud\OneDrive\!_munka\Revolution\StructuralParts\Brain\Inventor imported\BRpcbA\R149.iam
- C:\!_Dani\!_cloud\OneDrive\!_munka\Revolution\StructuralParts\Brain\Inventor imported\BRpcbA\R143.iam
- C:\!_Dani\!_cloud\OneDrive\!_munka\Revolution\StructuralParts\Brain\Inventor imported\BRpcbA\R140.iam
- C:\!_Dani\!_cloud\OneDrive\!_munka\Revolution\StructuralParts\Brain\Inventor imported\BRpcbA\R134.iam
- C:\!_Dani\!_cloud\OneDrive\!_munka\Revolution\StructuralParts\Brain\Inventor imported\BRpcbA\R120.iam
- C:\!_Dani\!_cloud\OneDrive\!_munka\Revolution\StructuralParts\Brain\Inventor imported\BRpcbA\R130.iam
- C:\!_Dani\!_cloud\OneDrive\!_munka\Revolution\StructuralParts\Brain\Inventor imported\BRpcbA\R124.iam
- C:\!_Dani\!_cloud\OneDrive\!_munka\Revolution\StructuralParts\Brain\Inventor imported\BRpcbA\R122.iam
- C:\!_Dani\!_cloud\OneDrive\!_munka\Revolution\StructuralParts\Brain\Inventor imported\BRpcbA\R121.iam
- C:\!_Dani\!_cloud\OneDrive\!_munka\Revolution\StructuralParts\Brain\Inventor imported\BRpcbA\R142.iam
- C:\!_Dani\!_cloud\OneDrive\!_munka\Revolution\StructuralParts\Brain\Inventor imported\BRpcbA\R146.iam
- C:\!_Dani\!_cloud\OneDrive\!_munka\Revolution\StructuralParts\Brain\Inventor imported\BRpcbA\R145.iam
- C:\!_Dani\!_cloud\OneDrive\!_munka\Revolution\StructuralParts\Brain\Inventor imported\BRpcbA\R87.iam
- C:\!_Dani\!_cloud\OneDrive\!_munka\Revolution\StructuralParts\Brain\Inventor imported\BRpcbA\R84.iam
- C:\!_Dani\!_cloud\OneDrive\!_munka\Revolution\StructuralParts\Brain\Inventor imported\BRpcbA\R83.iam
- C:\!_Dani\!_cloud\OneDrive\!_munka\Revolution\StructuralParts\Brain\Inventor imported\BRpcbA\R76.iam
- C:\!_Dani\!_cloud\OneDrive\!_munka\Revolution\StructuralParts\Brain\Inventor imported\BRpcbA\R112.iam
- C:\!_Dani\!_cloud\OneDrive\!_munka\Revolution\StructuralParts\Brain\Inventor imported\BRpcbA\R113.iam
- C:\!_Dani\!_cloud\OneDrive\!_munka\Revolution\StructuralParts\Brain\Inventor imported\BRpcbA\R73.iam
- C:\!_Dani\!_cloud\OneDrive\!_munka\Revolution\StructuralParts\Brain\Inventor imported\BRpcbA\R103.iam
- C:\!_Dani\!_cloud\OneDrive\!_munka\Revolution\StructuralParts\Brain\Inventor imported\BRpcbA\R102.iam
- C:\!_Dani\!_cloud\OneDrive\!_munka\Revolution\StructuralParts\Brain\Inventor imported\BRpcbA\R101.iam
- C:\!_Dani\!_cloud\OneDrive\!_munka\Revolution\StructuralParts\Brain\Inventor imported\BRpcbA\R62.iam
- C:\!_Dani\!_cloud\OneDrive\!_munka\Revolution\StructuralParts\Brain\Inventor imported\BRpcbA\R97.iam
- C:\!_Dani\!_cloud\OneDrive\!_munka\Revolution\StructuralParts\Brain\Inventor imported\BRpcbA\R60.iam
- C:\!_Dani\!_cloud\OneDrive\!_munka\Revolution\StructuralParts\Brain\Inventor imported\BRpcbA\R59.iam
- C:\!_Dani\!_cloud\OneDrive\!_munka\Revolution\StructuralParts\Brain\Inventor imported\BRpcbA\R91.iam
- C:\!_Dani\!_cloud\OneDrive\!_munka\Revolution\StructuralParts\Brain\Inventor imported\BRpcbA\R90.iam
- C:\!_Dani\!_cloud\OneDrive\!_munka\Revolution\StructuralParts\Brain\Inventor imported\BRpcbA\R77.iam
- C:\!_Dani\!_cloud\OneDrive\!_munka\Revolution\StructuralParts\Brain\Inventor imported\BRpcbA\R72.iam
- C:\!_Dani\!_cloud\OneDrive\!_munka\Revolution\StructuralParts\Brain\Inventor imported\BRpcbA\R53.iam
- C:\!_Dani\!_cloud\OneDrive\!_munka\Revolution\StructuralParts\Brain\Inventor imported\BRpcbA\R52.iam
- C:\!_Dani\!_cloud\OneDrive\!_munka\Revolution\StructuralParts\Brain\Inventor imported\BRpcbA\R86.iam
- C:\!_Dani\!_cloud\OneDrive\!_munka\Revolution\StructuralParts\Brain\Inventor imported\BRpcbA\R78.iam
- C:\!_Dani\!_cloud\OneDrive\!_munka\Revolution\StructuralParts\Brain\Inventor imported\BRpcbA\R75.iam
- C:\!_Dani\!_cloud\OneDrive\!_munka\Revolution\StructuralParts\Brain\Inventor imported\BRpcbA\R44.iam
- C:\!_Dani\!_cloud\OneDrive\!_munka\Revolution\StructuralParts\Brain\Inventor imported\BRpcbA\R40.iam
- C:\!_Dani\!_cloud\OneDrive\!_munka\Revolution\StructuralParts\Brain\Inventor imported\BRpcbA\R35.iam
- C:\!_Dani\!_cloud\OneDrive\!_munka\Revolution\StructuralParts\Brain\Inventor imported\BRpcbA\R14.iam
- C:\!_Dani\!_cloud\OneDrive\!_munka\Revolution\StructuralParts\Brain\Inventor imported\BRpcbA\R7.iam
- C:\!_Dani\!_cloud\OneDrive\!_munka\Revolution\StructuralParts\Brain\Inventor imported\BRpcbA\R18.iam
- C:\!_Dani\!_cloud\OneDrive\!_munka\Revolution\StructuralParts\Brain\Inventor imported\BRpcbA\R11.iam
- C:\!_Dani\!_cloud\OneDrive\!_munka\Revolution\StructuralParts\Brain\Inventor imported\BRpcbA\R1.iam
- C:\!_Dani\!_cloud\OneDrive\!_munka\Revolution\StructuralParts\Brain\Inventor imported\BRpcbA\R5.iam
- C:\!_Dani\!_cloud\OneDrive\!_munka\Revolution\StructuralParts\Brain\Inventor imported\BRpcbA\R4.iam
- C:\!_Dani\!_cloud\OneDrive\!_munka\Revolution\StructuralParts\Brain\Inventor imported\BRpcbA\R3.iam
- C:\!_Dani\!_cloud\OneDrive\!_munka\Revolution\StructuralParts\Brain\Inventor imported\BRpcbA\Q11.iam
- C:\!_Dani\!_cloud\OneDrive\!_munka\Revolution\StructuralParts\Brain\Inventor imported\BRpcbA\Q10.iam
- C:\!_Dani\!_cloud\OneDrive\!_munka\Revolution\StructuralParts\Brain\Inventor imported\BRpcbA\Q8.iam
- C:\!_Dani\!_cloud\OneDrive\!_munka\Revolution\StructuralParts\Brain\Inventor imported\BRpcbA\Q7.iam
- C:\!_Dani\!_cloud\OneDrive\!_munka\Revolution\StructuralParts\Brain\Inventor imported\BRpcbA\Q2.iam
- C:\!_Dani\!_cloud\OneDrive\!_munka\Revolution\StructuralParts\Brain\Inventor imported\BRpcbA\Q1.iam
- C:\!_Dani\!_cloud\OneDrive\!_munka\Revolution\StructuralParts\Brain\Inventor imported\BRpcbA\L3.iam
- C:\!_Dani\!_cloud\OneDrive\!_munka\Revolution\StructuralParts\Brain\Inventor imported\BRpcbA\L2.iam
- C:\!_Dani\!_cloud\OneDrive\!_munka\Revolution\StructuralParts\Brain\Inventor imported\BRpcbA\L1.iam
- C:\!_Dani\!_cloud\OneDrive\!_munka\Revolution\StructuralParts\Brain\Inventor imported\BRpcbA\FU18.iam
- C:\!_Dani\!_cloud\OneDrive\!_munka\Revolution\StructuralParts\Brain\Inventor imported\BRpcbA\FU17.iam
- C:\!_Dani\!_cloud\OneDrive\!_munka\Revolution\StructuralParts\Brain\Inventor imported\BRpcbA\FU12.iam
- C:\!_Dani\!_cloud\OneDrive\!_munka\Revolution\StructuralParts\Brain\Inventor imported\BRpcbA\FU11.iam
- C:\!_Dani\!_cloud\OneDrive\!_munka\Revolution\StructuralParts\Brain\Inventor imported\BRpcbA\FU2.iam
- C:\!_Dani\!_cloud\OneDrive\!_munka\Revolution\StructuralParts\Brain\Inventor imported\BRpcbA\FB8.iam
- C:\!_Dani\!_cloud\OneDrive\!_munka\Revolution\StructuralParts\Brain\Inventor imported\BRpcbA\FB3.iam
- C:\!_Dani\!_cloud\OneDrive\!_munka\Revolution\StructuralParts\Brain\Inventor imported\BRpcbA\FB2.iam
- C:\!_Dani\!_cloud\OneDrive\!_munka\Revolution\StructuralParts\Brain\Inventor imported\BRpcbA\D50.iam
- C:\!_Dani\!_cloud\OneDrive\!_munka\Revolution\StructuralParts\Brain\Inventor imported\BRpcbA\D49.iam
- C:\!_Dani\!_cloud\OneDrive\!_munka\Revolution\StructuralParts\Brain\Inventor imported\BRpcbA\D47.iam
- C:\!_Dani\!_cloud\OneDrive\!_munka\Revolution\StructuralParts\Brain\Inventor imported\BRpcbA\D45.iam
- C:\!_Dani\!_cloud\OneDrive\!_munka\Revolution\StructuralParts\Brain\Inventor imported\BRpcbA\D44.iam
- C:\!_Dani\!_cloud\OneDrive\!_munka\Revolution\StructuralParts\Brain\Inventor imported\BRpcbA\D30.iam
- C:\!_Dani\!_cloud\OneDrive\!_munka\Revolution\StructuralParts\Brain\Inventor imported\BRpcbA\D29.iam
- C:\!_Dani\!_cloud\OneDrive\!_munka\Revolution\StructuralParts\Brain\Inventor imported\BRpcbA\D25.iam
- C:\!_Dani\!_cloud\OneDrive\!_munka\Revolution\StructuralParts\Brain\Inventor imported\BRpcbA\D16.iam
- C:\!_Dani\!_cloud\OneDrive\!_munka\Revolution\StructuralParts\Brain\Inventor imported\BRpcbA\D2.iam
- C:\!_Dani\!_cloud\OneDrive\!_munka\Revolution\StructuralParts\Brain\Inventor imported\BRpcbA\CON8.iam
- C:\!_Dani\!_cloud\OneDrive\!_munka\Revolution\StructuralParts\Brain\Inventor imported\BRpcbA\CON6.iam
- C:\!_Dani\!_cloud\OneDrive\!_munka\Revolution\StructuralParts\Brain\Inventor imported\BRpcbA\CON7.iam
- C:\!_Dani\!_cloud\OneDrive\!_munka\Revolution\StructuralParts\Brain\Inventor imported\BRpcbA\CON5.iam
- C:\!_Dani\!_cloud\OneDrive\!_munka\Revolution\StructuralParts\Brain\Inventor imported\BRpcbA\CON4.iam
- C:\!_Dani\!_cloud\OneDrive\!_munka\Revolution\StructuralParts\Brain\Inventor imported\BRpcbA\CON3.iam
- C:\!_Dani\!_cloud\OneDrive\!_munka\Revolution\StructuralParts\Brain\Inventor imported\BRpcbA\C82.iam
- C:\!_Dani\!_cloud\OneDrive\!_munka\Revolution\StructuralParts\Brain\Inventor imported\BRpcbA\C38.iam
- C:\!_Dani\!_cloud\OneDrive\!_munka\Revolution\StructuralParts\Brain\Inventor imported\BRpcbA\C106.iam
- C:\!_Dani\!_cloud\OneDrive\!_munka\Revolution\StructuralParts\Brain\Inventor imported\BRpcbA\C105.iam
- C:\!_Dani\!_cloud\OneDrive\!_munka\Revolution\StructuralParts\Brain\Inventor imported\BRpcbA\C107.iam
- C:\!_Dani\!_cloud\OneDrive\!_munka\Revolution\StructuralParts\Brain\Inventor imported\BRpcbA\C99.iam
- C:\!_Dani\!_cloud\OneDrive\!_munka\Revolution\StructuralParts\Brain\Inventor imported\BRpcbA\C98.iam
- C:\!_Dani\!_cloud\OneDrive\!_munka\Revolution\StructuralParts\Brain\Inventor imported\BRpcbA\C109.iam
- C:\!_Dani\!_cloud\OneDrive\!_munka\Revolution\StructuralParts\Brain\Inventor imported\BRpcbA\C93.iam
- C:\!_Dani\!_cloud\OneDrive\!_munka\Revolution\StructuralParts\Brain\Inventor imported\BRpcbA\C92.iam
- C:\!_Dani\!_cloud\OneDrive\!_munka\Revolution\StructuralParts\Brain\Inventor imported\BRpcbA\C83.iam
- C:\!_Dani\!_cloud\OneDrive\!_munka\Revolution\StructuralParts\Brain\Inventor imported\BRpcbA\C95.iam
- C:\!_Dani\!_cloud\OneDrive\!_munka\Revolution\StructuralParts\Brain\Inventor imported\BRpcbA\C49.iam
- C:\!_Dani\!_cloud\OneDrive\!_munka\Revolution\StructuralParts\Brain\Inventor imported\BRpcbA\C89.iam
- C:\!_Dani\!_cloud\OneDrive\!_munka\Revolution\StructuralParts\Brain\Inventor imported\BRpcbA\C87.iam
- C:\!_Dani\!_cloud\OneDrive\!_munka\Revolution\StructuralParts\Brain\Inventor imported\BRpcbA\C44.iam
- C:\!_Dani\!_cloud\OneDrive\!_munka\Revolution\StructuralParts\Brain\Inventor imported\BRpcbA\C43.iam
- C:\!_Dani\!_cloud\OneDrive\!_munka\Revolution\StructuralParts\Brain\Inventor imported\BRpcbA\C96.iam
- C:\!_Dani\!_cloud\OneDrive\!_munka\Revolution\StructuralParts\Brain\Inventor imported\BRpcbA\C94.iam
- C:\!_Dani\!_cloud\OneDrive\!_munka\Revolution\StructuralParts\Brain\Inventor imported\BRpcbA\C68.iam
- C:\!_Dani\!_cloud\OneDrive\!_munka\Revolution\StructuralParts\Brain\Inventor imported\BRpcbA\C67.iam
- C:\!_Dani\!_cloud\OneDrive\!_munka\Revolution\StructuralParts\Brain\Inventor imported\BRpcbA\C66.iam
- C:\!_Dani\!_cloud\OneDrive\!_munka\Revolution\StructuralParts\Brain\Inventor imported\BRpcbA\C65.iam
- C:\!_Dani\!_cloud\OneDrive\!_munka\Revolution\StructuralParts\Brain\Inventor imported\BRpcbA\C62.iam
- C:\!_Dani\!_cloud\OneDrive\!_munka\Revolution\StructuralParts\Brain\Inventor imported\BRpcbA\C61.iam
- C:\!_Dani\!_cloud\OneDrive\!_munka\Revolution\StructuralParts\Brain\Inventor imported\BRpcbA\C60.iam
- C:\!_Dani\!_cloud\OneDrive\!_munka\Revolution\StructuralParts\Brain\Inventor imported\BRpcbA\C59.iam
- C:\!_Dani\!_cloud\OneDrive\!_munka\Revolution\StructuralParts\Brain\Inventor imported\BRpcbA\C57.iam
- C:\!_Dani\!_cloud\OneDrive\!_munka\Revolution\StructuralParts\Brain\Inventor imported\BRpcbA\C56.iam
- C:\!_Dani\!_cloud\OneDrive\!_munka\Revolution\StructuralParts\Brain\Inventor imported\BRpcbA\C69.iam
- C:\!_Dani\!_cloud\OneDrive\!_munka\Revolution\StructuralParts\Brain\Inventor imported\BRpcbA\C54.iam
- C:\!_Dani\!_cloud\OneDrive\!_munka\Revolution\StructuralParts\Brain\Inventor imported\BRpcbA\C52.iam
- C:\!_Dani\!_cloud\OneDrive\!_munka\Revolution\StructuralParts\Brain\Inventor imported\BRpcbA\C50.iam
- C:\!_Dani\!_cloud\OneDrive\!_munka\Revolution\StructuralParts\Brain\Inventor imported\BRpcbA\C41.iam
- C:\!_Dani\!_cloud\OneDrive\!_munka\Revolution\StructuralParts\Brain\Inventor imported\BRpcbA\C17.iam
- C:\!_Dani\!_cloud\OneDrive\!_munka\Revolution\StructuralParts\Brain\Inventor imported\BRpcbA\C16.iam
- C:\!_Dani\!_cloud\OneDrive\!_munka\Revolution\StructuralParts\Brain\Inventor imported\BRpcbA\C14.iam
- C:\!_Dani\!_cloud\OneDrive\!_munka\Revolution\StructuralParts\Brain\Inventor imported\BRpcbA\C15.iam
- C:\!_Dani\!_cloud\OneDrive\!_munka\Revolution\StructuralParts\Brain\Inventor imported\BRpcbA\C13.iam
- C:\!_Dani\!_cloud\OneDrive\!_munka\Revolution\StructuralParts\Brain\Inventor imported\BRpcbA\C12.iam
- C:\!_Dani\!_cloud\OneDrive\!_munka\Revolution\StructuralParts\Brain\Inventor imported\BRpcbA\C11.iam
- C:\!_Dani\!_cloud\OneDrive\!_munka\Revolution\StructuralParts\Brain\Inventor imported\BRpcbA\C10.iam
- C:\!_Dani\!_cloud\OneDrive\!_munka\Revolution\StructuralParts\Brain\Inventor imported\BRpcbA\C9.iam
- C:\!_Dani\!_cloud\OneDrive\!_munka\Revolution\StructuralParts\Brain\Inventor imported\BRpcbA\C8.iam
- C:\!_Dani\!_cloud\OneDrive\!_munka\Revolution\StructuralParts\Brain\Inventor imported\BRpcbA\C7.iam
- C:\!_Dani\!_cloud\OneDrive\!_munka\Revolution\StructuralParts\Brain\Inventor imported\BRpcbA\C6.iam
- C:\!_Dani\!_cloud\OneDrive\!_munka\Revolution\StructuralParts\Brain\Inventor imported\BRpcbA\C5.iam
- C:\!_Dani\!_cloud\OneDrive\!_munka\Revolution\StructuralParts\Brain\Inventor imported\BRpcbA\C4.iam
- C:\!_Dani\!_cloud\OneDrive\!_munka\Revolution\StructuralParts\Brain\Inventor imported\BRpcbA\C3.iam
- C:\!_Dani\!_cloud\OneDrive\!_munka\Revolution\StructuralParts\Brain\Inventor imported\BRpcbA\C1.iam
## Components (427 placed, 427 different names)
1. Board_2 [sub-assembly]
2. R177_4 [sub-assembly]
3. CON1_6 [sub-assembly]
4. R81_8 [sub-assembly]
5. C45_10 [sub-assembly]
6. U4_12 [sub-assembly]
7. D37_14 [sub-assembly]
8. D33_16 [sub-assembly]
9. D32_18 [sub-assembly]
10. C48_20 [sub-assembly]
11. C47_22 [sub-assembly]
12. D31_24 [sub-assembly]
13. C46_26 [sub-assembly]
14. R82_28 [sub-assembly]
15. R26_30 [sub-assembly]
16. C20_32 [sub-assembly]
17. U2_34 [sub-assembly]
18. D9_36 [sub-assembly]
19. D5_38 [sub-assembly]
20. D4_40 [sub-assembly]
21. C23_42 [sub-assembly]
22. C22_44 [sub-assembly]
23. D1_46 [sub-assembly]
24. C21_48 [sub-assembly]
25. R27_50 [sub-assembly]
26. R180_52 [sub-assembly]
27. R109_54 [sub-assembly]
28. R71_56 [sub-assembly]
29. D72_58 [sub-assembly]
30. Q4_60 [sub-assembly]
31. R176_62 [sub-assembly]
32. R175_64 [sub-assembly]
33. R174_66 [sub-assembly]
34. R173_68 [sub-assembly]
35. R172_70 [sub-assembly]
36. R171_72 [sub-assembly]
37. R170_74 [sub-assembly]
38. R169_76 [sub-assembly]
39. R168_78 [sub-assembly]
40. R167_80 [sub-assembly]
41. R166_82 [sub-assembly]
42. R165_84 [sub-assembly]
43. R80_86 [sub-assembly]
44. R79_88 [sub-assembly]
45. R67_90 [sub-assembly]
46. R66_92 [sub-assembly]
47. R51_94 [sub-assembly]
48. R50_96 [sub-assembly]
49. R39_98 [sub-assembly]
50. R38_100 [sub-assembly]
51. R23_102 [sub-assembly]
52. R22_104 [sub-assembly]
53. R9_106 [sub-assembly]
54. R8_108 [sub-assembly]
55. FB1_110 [sub-assembly]
56. C2_112 [sub-assembly]
57. FU1_114 [sub-assembly]
58. C97_116 [sub-assembly]
59. U16_118 [sub-assembly]
60. U14_120 [sub-assembly]
61. U8_123 [sub-assembly]
62. U6_125 [sub-assembly]
63. R161_127 [sub-assembly]
64. R150_129 [sub-assembly]
65. R127_131 [sub-assembly]
66. R118_133 [sub-assembly]
67. R116_135 [sub-assembly]
68. R115_137 [sub-assembly]
69. R114_139 [sub-assembly]
70. R111_141 [sub-assembly]
71. R110_143 [sub-assembly]
72. R106_145 [sub-assembly]
73. R105_147 [sub-assembly]
74. R99_149 [sub-assembly]
75. R98_151 [sub-assembly]
76. R95_153 [sub-assembly]
77. R92_155 [sub-assembly]
78. R89_157 [sub-assembly]
79. R88_159 [sub-assembly]
80. R74_161 [sub-assembly]
81. R68_163 [sub-assembly]
82. R54_165 [sub-assembly]
83. R47_167 [sub-assembly]
84. R46_169 [sub-assembly]
85. R45_171 [sub-assembly]
86. R41_173 [sub-assembly]
87. R32_175 [sub-assembly]
88. R31_177 [sub-assembly]
89. R29_179 [sub-assembly]
90. R28_181 [sub-assembly]
91. R19_183 [sub-assembly]
92. R15_185 [sub-assembly]
93. R12_187 [sub-assembly]
94. R2_189 [sub-assembly]
95. L4_191 [sub-assembly]
96. FU21_194 [sub-assembly]
97. FB11_196 [sub-assembly]
98. FB9_198 [sub-assembly]
99. FB7_200 [sub-assembly]
100. FB5_202 [sub-assembly]
101. D55_205 [sub-assembly]
102. D53_208 [sub-assembly]
103. D52_210 [sub-assembly]
104. D51_212 [sub-assembly]
105. D48_215 [sub-assembly]
106. D43_218 [sub-assembly]
107. D42_220 [sub-assembly]
108. D38_222 [sub-assembly]
109. D26_224 [sub-assembly]
110. D15_226 [sub-assembly]
111. D11_228 [sub-assembly]
112. D7_230 [sub-assembly]
113. D6_232 [sub-assembly]
114. D3_234 [sub-assembly]
115. C117_236 [sub-assembly]
116. C116_238 [sub-assembly]
117. C115_240 [sub-assembly]
118. C114_242 [sub-assembly]
119. C113_244 [sub-assembly]
120. C101_246 [sub-assembly]
121. C91_248 [sub-assembly]
122. C85_250 [sub-assembly]
123. C80_252 [sub-assembly]
124. C78_254 [sub-assembly]
125. C77_256 [sub-assembly]
126. C76_258 [sub-assembly]
127. C75_260 [sub-assembly]
128. C72_262 [sub-assembly]
129. C70_264 [sub-assembly]
130. C58_266 [sub-assembly]
131. C55_268 [sub-assembly]
132. C37_270 [sub-assembly]
133. C32_272 [sub-assembly]
134. C29_274 [sub-assembly]
135. R108_276 [sub-assembly]
136. R107_278 [sub-assembly]
137. D46_280 [sub-assembly]
138. C71_282 [sub-assembly]
139. D71_284 [sub-assembly]
140. D70_286 [sub-assembly]
141. D69_288 [sub-assembly]
142. D68_290 [sub-assembly]
143. D66_292 [sub-assembly]
144. D65_294 [sub-assembly]
145. D64_296 [sub-assembly]
146. D61_298 [sub-assembly]
147. D60_300 [sub-assembly]
148. D17_302 [sub-assembly]
149. R148_304 [sub-assembly]
150. D58_306 [sub-assembly]
151. D56_308 [sub-assembly]
152. D24_310 [sub-assembly]
153. D63_312 [sub-assembly]
154. D67_314 [sub-assembly]
155. Q16_316 [sub-assembly]
156. Q17_318 [sub-assembly]
157. R153_320 [sub-assembly]
158. R156_322 [sub-assembly]
159. R139_324 [sub-assembly]
160. R144_326 [sub-assembly]
161. R141_328 [sub-assembly]
162. Q15_330 [sub-assembly]
163. Q14_332 [sub-assembly]
164. D62_334 [sub-assembly]
165. D59_336 [sub-assembly]
166. D54_338 [sub-assembly]
167. D57_340 [sub-assembly]
168. Q12_342 [sub-assembly]
169. Q13_344 [sub-assembly]
170. R131_346 [sub-assembly]
171. R132_348 [sub-assembly]
172. C42_350 [sub-assembly]
173. C33_352 [sub-assembly]
174. R58_354 [sub-assembly]
175. R55_356 [sub-assembly]
176. R48_358 [sub-assembly]
177. R34_360 [sub-assembly]
178. R49_362 [sub-assembly]
179. Q5_364 [sub-assembly]
180. FU8_366 [sub-assembly]
181. FU7_368 [sub-assembly]
182. D36_370 [sub-assembly]
183. D35_372 [sub-assembly]
184. D34_374 [sub-assembly]
185. C63_376 [sub-assembly]
186. C36_378 [sub-assembly]
187. C35_380 [sub-assembly]